# Autodesk Inventor assembly: am-3232-731 + am-0143
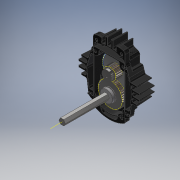
[picture p0: Inventor's stored thumbnail of the model, 180x180]
Saved by Autodesk Inventor 2018 (Build 220112000, 112)
## iProperties
Created: 2018-11-10
Part Number: am-3232-731 + am-0143
Document SubType Name: Assembly
Designer: TODD D MILLER
Description: TB Micro/Mini gearbox 7.31:1 ratio  AL cl; long hex -1in shaft; plate-none
Mass: 3657.84 g
Surface Area: 2662.8 cm^2
Volume: 1052.52 cm^3
Density: 3.47531 g/cm^3
Vendor: AndyMark
RuleStatus: InUse
Author: TODD D MILLER
## Documents named in this file (29)
- G:\FRC\CAD Library\GEARBOX\Toughbox gearbox 731 Mini-Micro for assembly (iLogic).iam
- G:\FRC\CAD Library\GEARBOX\gearbox - ToughBox mini\am-0650 - Toughbox Mini Housing.ipt
- G:\FRC\CAD Library\SHAFTS\BEARINGS\am-0516 - 0375 in id bearing, shielded (R6ZZ).ipt
- G:\FRC\CAD Library\GEARBOX\SHAFTS\Toughbox Small 375 Hex Shaft (am-0152).ipt
- G:\FRC\CAD Library\GEARS\am-0149 - 50T Toughbox Large Cluster Gear - steel.ipt
- G:\FRC\CAD Library\BEARINGS\FR6ZZ Bearing_smart.ipt
- G:\FRC\CAD Library\SHAFTS\RINGS\External Klipring for 500 shaft (am-0206).ipt
- G:\FRC\CAD Library\GEARS\am-0143 - 50T Toughbox Large Cluster Gear - AL.ipt
- G:\FRC\CAD Library\GEARBOX\gearbox - ToughBox mini\ToughBox mini short 500 round shaft sub-assy.iam
- G:\FRC\CAD Library\GEARBOX\gearbox - ToughBox mini\ToughBox mini short 500 hex shaft sub-assy.iam
- G:\FRC\CAD Library\GEARBOX\gearbox - ToughBox mini\ToughBox mini long 500 round shaft sub-assy.iam
- G:\FRC\CAD Library\GEARBOX\gearbox - ToughBox mini\ToughBox mini long 500 hex shaft sub-assy.iam
- G:\FRC\CAD Library\GEARBOX\gearbox - ToughBox mini\ToughBox mini 595 gear sub-assy.iam
- G:\FRC\CAD Library\GEARBOX\gearbox - ToughBox mini\ToughBox mini 731 gear sub-assy.iam
- G:\FRC\CAD Library\GEARBOX\gearbox - ToughBox mini\ToughBox mini 845 steel gear sub-assy.iam
- G:\FRC\CAD Library\GEARBOX\gearbox - ToughBox mini\ToughBox mini 845 AL gear sub-assy.iam
- G:\FRC\CAD Library\GEARBOX\gearbox - ToughBox mini\ToughBox mini 1071 steel gear sub-assy.iam
- G:\FRC\CAD Library\GEARBOX\gearbox - ToughBox mini\ToughBox mini 1071 AL gear sub-assy.iam
- G:\FRC\CAD Library\GEARBOX\gearbox - ToughBox mini\ToughBox mini 1275 steel gear sub-assy.iam
- G:\FRC\CAD Library\GEARBOX\gearbox - ToughBox mini\ToughBox mini 1275 AL gear sub-assy.iam
- G:\FRC\CAD Library\GEARBOX\am-2230+TM+Flat+Shaft+Plate.ipt
- G:\FRC\CAD Library\GEARBOX\TB Mini flat face plate.ipt
- G:\FRC\CAD Library\GEARBOX\am-0647 - TM ANGLED Shaft Plate.ipt
- G:\FRC\CAD Library\GEARBOX\gearbox - ToughBox mini\ToughBox mini long 500 hex shaft sub-assy (short 1in).iam
- G:\FRC\CAD Library\GEARBOX\TB Mini shell mounting screws.iam
- G:\FRC\CAD Library\GEARBOX\am-3157 TB Micro housing.ipt
- G:\FRC\CAD Library\GEARBOX\am-3229 TB Micro flat plate.ipt
- G:\FRC\CAD Library\GEARBOX\am-3228 TB Micro angled plate.ipt
- G:\FRC\CAD Library\GEARBOX\TB Micro shell mounting screws.iam
## Components (29 placed, 28 different names)
1. am-0650 - Toughbox Mini Housing:1 — Flush:1, Mate:1, Flush:2, Mate:3, Mate:4, Mate:5, Insert:1, Insert:2, Flush:3, Insert:49, Insert:53, Insert:54
2. TB Mini shell mounting screws:1 [sub-assembly]
3. am-3157 TB Micro housing:1 — Mate:24, Mate:25, Flush:8
4. am-3229 TB Micro flat plate:1
5. am-3228 TB Micro angled plate:1
6. TB Micro shell mounting screws:1 [sub-assembly]
7. External Klipring for 500 shaft (am-0206):1
8. am-0516 - 0375 in id bearing, shielded (R6ZZ):2 — Insert:1, Insert:3, Insert:4, Insert:5
9. Toughbox Small 375 Hex Shaft (am-0152):1 — Insert:3, Mate:6
10. am-0149 - 50T Toughbox Large Cluster Gear - steel:1 — Insert:4
11. am-0143 - 50T Toughbox Large Cluster Gear - AL:1 — Insert:5
12. am-0516 - 0375 in id bearing, shielded (R6ZZ):1 — Insert:2, Insert:55
13. FR6ZZ Bearing_smart:1 — Mate:6, Flush:3
14. ToughBox mini long 500 hex shaft sub-assy (short 1in):1 [sub-assembly] — Insert:55
15. ToughBox mini short 500 round shaft sub-assy:1 [sub-assembly]
16. ToughBox mini short 500 hex shaft sub-assy:1 [sub-assembly]
17. ToughBox mini long 500 round shaft sub-assy:1 [sub-assembly]
18. ToughBox mini long 500 hex shaft sub-assy:1 [sub-assembly]
19. ToughBox mini 595 gear sub-assy:1 [sub-assembly]
20. ToughBox mini 731 gear sub-assy:1 [sub-assembly]
21. ToughBox mini 845 steel gear sub-assy:1 [sub-assembly]
22. ToughBox mini 845 AL gear sub-assy:1 [sub-assembly]
23. ToughBox mini 1071 steel gear sub-assy:1 [sub-assembly]
24. ToughBox mini 1071 AL gear sub-assy:1 [sub-assembly]
25. ToughBox mini 1275 steel gear sub-assy:1 [sub-assembly]
26. ToughBox mini 1275 AL gear sub-assy:1 [sub-assembly]
27. am-2230+TM+Flat+Shaft+Plate:1 — Insert:49
28. TB Mini flat face plate:1
29. am-0647 - TM ANGLED Shaft Plate:1 — Insert:53, Insert:54
## Relationships (74: Insert 52, Mate 14, Flush 8)
- Flush:1: am-0650 - Toughbox Mini Housing:1
- Mate:1: am-0650 - Toughbox Mini Housing:1
- Mate:2
- Flush:2: am-0650 - Toughbox Mini Housing:1
- Mate:3: am-0650 - Toughbox Mini Housing:1
- Mate:4: am-0650 - Toughbox Mini Housing:1
- Mate:5: am-0650 - Toughbox Mini Housing:1
- Insert:1: am-0650 - Toughbox Mini Housing:1 ↔ am-0516 - 0375 in id bearing, shielded (R6ZZ):2
- Insert:2: am-0650 - Toughbox Mini Housing:1 ↔ am-0516 - 0375 in id bearing, shielded (R6ZZ):1
- Insert:3: am-0516 - 0375 in id bearing, shielded (R6ZZ):2 ↔ Toughbox Small 375 Hex Shaft (am-0152):1
- Insert:4: am-0516 - 0375 in id bearing, shielded (R6ZZ):2 ↔ am-0149 - 50T Toughbox Large Cluster Gear - steel:1
- Insert:5: am-0516 - 0375 in id bearing, shielded (R6ZZ):2 ↔ am-0143 - 50T Toughbox Large Cluster Gear - AL:1
- Mate:6: Toughbox Small 375 Hex Shaft (am-0152):1 ↔ FR6ZZ Bearing_smart:1
- Flush:3: am-0650 - Toughbox Mini Housing:1 ↔ FR6ZZ Bearing_smart:1
- [Insert]: Toughbox Small 375 Hex Shaft (am-0152):1 ↔ ToughBox mini 1071 AL gear sub-assy:1
- [Insert]: am-0516 - 0375 in id bearing, shielded (R6ZZ):1 ↔ ToughBox mini short 500 round shaft sub-assy:1
- [Insert]: am-0516 - 0375 in id bearing, shielded (R6ZZ):1 ↔ ToughBox mini short 500 hex shaft sub-assy:1
- [Insert]: am-0516 - 0375 in id bearing, shielded (R6ZZ):1 ↔ ToughBox mini long 500 round shaft sub-assy:1
- [Insert]: am-0516 - 0375 in id bearing, shielded (R6ZZ):1 ↔ ToughBox mini long 500 hex shaft sub-assy:1
- [Flush]: am-0650 - Toughbox Mini Housing:1 ↔ ToughBox mini short 500 round shaft sub-assy:1
- [Flush]: am-0650 - Toughbox Mini Housing:1 ↔ ToughBox mini short 500 hex shaft sub-assy:1
- [Mate]: ToughBox mini short 500 round shaft sub-assy:1
- [Mate]: ToughBox mini short 500 hex shaft sub-assy:1
- [Insert] (3.175 mm): am-0650 - Toughbox Mini Housing:1 ↔ TB Mini shell mounting screws:1
- [Insert] (3.175 mm): am-0650 - Toughbox Mini Housing:1 ↔ TB Mini shell mounting screws:1
- [Insert] (3.175 mm): am-0650 - Toughbox Mini Housing:1 ↔ TB Mini shell mounting screws:1
- [Insert] (3.175 mm): am-0650 - Toughbox Mini Housing:1 ↔ TB Mini shell mounting screws:1
- [Insert]: am-0650 - Toughbox Mini Housing:1 ↔ TB Mini shell mounting screws:1
- [Insert]: am-0650 - Toughbox Mini Housing:1 ↔ TB Mini shell mounting screws:1
- [Insert]: am-0650 - Toughbox Mini Housing:1 ↔ TB Mini shell mounting screws:1
- [Insert]: am-0650 - Toughbox Mini Housing:1 ↔ TB Mini shell mounting screws:1
- [Insert]: External Klipring for 500 shaft (am-0206):1 ↔ ToughBox mini 1071 steel gear sub-assy:1
- [Insert]: External Klipring for 500 shaft (am-0206):1 ↔ ToughBox mini 1275 AL gear sub-assy:1
- [Insert]: FR6ZZ Bearing_smart:1 ↔ ToughBox mini 1275 AL gear sub-assy:1
- [Insert]: External Klipring for 500 shaft (am-0206):1 ↔ ToughBox mini 1275 steel gear sub-assy:1
- [Insert]: External Klipring for 500 shaft (am-0206):1 ↔ ToughBox mini 845 steel gear sub-assy:1
- [Insert]: FR6ZZ Bearing_smart:1 ↔ ToughBox mini 845 AL gear sub-assy:1
- [Insert]: External Klipring for 500 shaft (am-0206):1 ↔ ToughBox mini 1071 AL gear sub-assy:1
- [Insert]: External Klipring for 500 shaft (am-0206):1 ↔ ToughBox mini 845 AL gear sub-assy:1
- [Insert]: External Klipring for 500 shaft (am-0206):1 ↔ ToughBox mini 731 gear sub-assy:1
- [Insert]: Toughbox Small 375 Hex Shaft (am-0152):1 ↔ ToughBox mini 731 gear sub-assy:1
- [Insert]: Toughbox Small 375 Hex Shaft (am-0152):1 ↔ ToughBox mini 595 gear sub-assy:1
- [Insert]: External Klipring for 500 shaft (am-0206):1 ↔ ToughBox mini 595 gear sub-assy:1
- [Flush]: am-0650 - Toughbox Mini Housing:1 ↔ ToughBox mini long 500 hex shaft sub-assy:1
- [Mate]: ToughBox mini long 500 hex shaft sub-assy:1
- [Flush]: am-0650 - Toughbox Mini Housing:1 ↔ ToughBox mini long 500 round shaft sub-assy:1
- [Mate]: ToughBox mini long 500 round shaft sub-assy:1
- [Insert]: FR6ZZ Bearing_smart:1 ↔ ToughBox mini 845 steel gear sub-assy:1
- [Insert]: FR6ZZ Bearing_smart:1 ↔ ToughBox mini 1071 steel gear sub-assy:1
- [Insert]: FR6ZZ Bearing_smart:1 ↔ ToughBox mini 1275 steel gear sub-assy:1
- Insert:49: am-0650 - Toughbox Mini Housing:1 ↔ am-2230+TM+Flat+Shaft+Plate:1
- [Insert]: TB Mini shell mounting screws:1 ↔ am-2230+TM+Flat+Shaft+Plate:1
- [Insert]: TB Mini shell mounting screws:1 ↔ TB Mini flat face plate:1
- [Insert]: TB Mini shell mounting screws:1 ↔ TB Mini flat face plate:1
- Insert:53: am-0650 - Toughbox Mini Housing:1 ↔ am-0647 - TM ANGLED Shaft Plate:1
- Insert:54: am-0650 - Toughbox Mini Housing:1 ↔ am-0647 - TM ANGLED Shaft Plate:1
- Insert:55: am-0516 - 0375 in id bearing, shielded (R6ZZ):1 ↔ ToughBox mini long 500 hex shaft sub-assy (short 1in):1
- [Insert] (3.175 mm): am-3157 TB Micro housing:1 ↔ TB Micro shell mounting screws:1
- [Insert] (3.175 mm): am-3157 TB Micro housing:1 ↔ TB Micro shell mounting screws:1
- [Insert] (3.175 mm): am-3157 TB Micro housing:1 ↔ TB Micro shell mounting screws:1
- [Insert] (3.175 mm): am-3157 TB Micro housing:1 ↔ TB Micro shell mounting screws:1
- [Insert]: am-3157 TB Micro housing:1 ↔ TB Micro shell mounting screws:1
- [Insert]: am-3157 TB Micro housing:1 ↔ TB Micro shell mounting screws:1
- [Insert]: am-3157 TB Micro housing:1 ↔ TB Micro shell mounting screws:1
- [Insert]: am-3157 TB Micro housing:1 ↔ TB Micro shell mounting screws:1
- [Mate]: am-3157 TB Micro housing:1 ↔ am-3228 TB Micro angled plate:1
- [Mate]: am-3157 TB Micro housing:1 ↔ am-3229 TB Micro flat plate:1
- [Insert]: am-3228 TB Micro angled plate:1 ↔ TB Micro shell mounting screws:1
- [Insert]: am-3228 TB Micro angled plate:1 ↔ TB Micro shell mounting screws:1
- [Insert]: am-3229 TB Micro flat plate:1 ↔ TB Micro shell mounting screws:1
- [Insert]: am-3229 TB Micro flat plate:1 ↔ TB Micro shell mounting screws:1
- Mate:24: am-3157 TB Micro housing:1
- Mate:25: am-3157 TB Micro housing:1
- Flush:8: am-3157 TB Micro housing:1
## Named parameters: plate_thickness = 3.175 mm
